# Autodesk Inventor assembly: chumacera_rodaje_grande
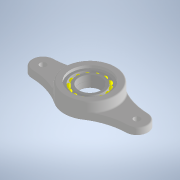
[picture p0: Inventor's stored thumbnail of the model, 180x180]
Saved by Autodesk Inventor 2021 (Build 250183000, 183)
## iProperties
Created: 2021-10-11
Part Number: chumacera_rodaje_grande
Document SubType Name: Assembly
Designer: arthu
Author: arthu
## Documents named in this file (3)
- C:\Users\arthu\OneDrive\Escritorio\Faja\chumacera_rodaje_grande.iam
- C:\Users\arthu\OneDrive\Escritorio\Faja\chumacera_grande.ipt
- C:\Users\arthu\OneDrive\Escritorio\Faja\AIS2021\SKF_16007.iam
## Components (3 placed, 2 different names)
1. chumacera_grande:1 — De rotación:1
2. SKF_16007:1 [sub-assembly] — De rotación:1, De rotación:2
3. SKF_16007:2 [sub-assembly] — De rotación:2
## Relationships (2: RevoluteJoint 2)
- De rotación:1 [RevoluteJoint] (4 mm): chumacera_grande:1 ↔ SKF_16007:1
- De rotación:2 [RevoluteJoint]: SKF_16007:1 ↔ SKF_16007:2
